# Autodesk Inventor assembly: Nozzle Master Sketch
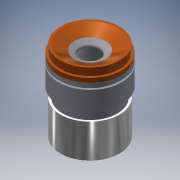
[picture p0: Inventor's stored thumbnail of the model, 180x180]
Saved by Autodesk Inventor 2017 (Build 210142000, 142)
## iProperties
Created: 2016-07-25
Part Number: Nozzle Master Sketch
Document SubType Name: Assembly
Designer: Bill
Author: Bill
## Documents named in this file (6)
- D:\Triton_Rocket_Club\Propulsion\Launches\8-inch-flight\Design\CAD\Nozzle\trunk\Nozzle Master Sketch.iam
- D:\Triton_Rocket_Club\Propulsion\Launches\8-inch-flight\Design\CAD\Nozzle\trunk\Graphite Master Sketch.ipt
- D:\Triton_Rocket_Club\Propulsion\Launches\8-inch-flight\Design\CAD\Nozzle\trunk\Phenolic Master Sketch.ipt
- D:\Triton_Rocket_Club\Propulsion\Launches\8-inch-flight\Design\CAD\Nozzle\trunk\Carrier Master Sketch.ipt
- D:\Triton_Rocket_Club\Propulsion\Launches\8-inch-flight\Design\CAD\Nozzle\trunk\Retainer Master Sketch.ipt
- D:\Triton_Rocket_Club\Propulsion\Launches\8-inch-flight\Design\CAD\Nozzle\trunk\Skirt Master Sketch.ipt
## Components (5 placed, 5 different names)
1. Graphite Master Sketch:1 — Mate:1
2. Phenolic Master Sketch:1 — Mate:1, Mate:2, Mate:5, Mate:7
3. Carrier Master Sketch:1 — Mate:2, Mate:3, Mate:4, Mate:5, Mate:6, Mate:7, Mate:8
4. Retainer Master Sketch:1 — Mate:3, Mate:4
5. Skirt Master Sketch:1 — Mate:6, Mate:8
## Relationships (8: Mate 8)
- Mate:1: Graphite Master Sketch:1 ↔ Phenolic Master Sketch:1
- Mate:2: Phenolic Master Sketch:1 ↔ Carrier Master Sketch:1
- Mate:3: Carrier Master Sketch:1 ↔ Retainer Master Sketch:1
- Mate:4: Carrier Master Sketch:1 ↔ Retainer Master Sketch:1
- Mate:5: Phenolic Master Sketch:1 ↔ Carrier Master Sketch:1
- Mate:6: Carrier Master Sketch:1 ↔ Skirt Master Sketch:1
- Mate:7: Phenolic Master Sketch:1 ↔ Carrier Master Sketch:1
- Mate:8: Carrier Master Sketch:1 ↔ Skirt Master Sketch:1
